# Autodesk Inventor assembly: gear_assembly
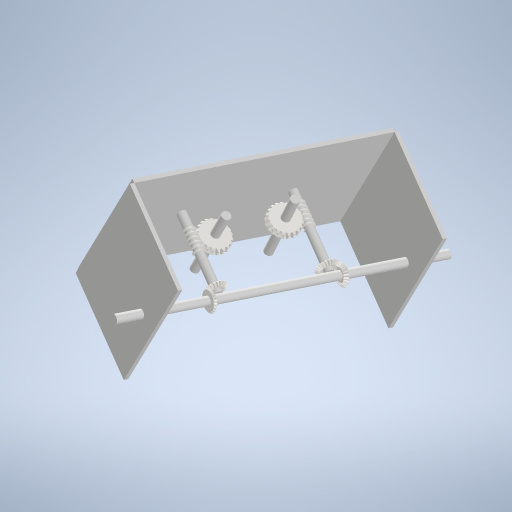
[picture p0: Inventor's stored thumbnail of the model, 512x512]
Saved by Autodesk Inventor 2023 (Build 270158000, 158)
## iProperties
Created: 2023-02-08
Part Number: gear_assembly
Document SubType Name: Assembly
Designer: Nikhil
Author: Nikhil
## Documents named in this file (8)
- C:\Users\Nikhil\Downloads\gear_assembly.iam
- C:\Users\Nikhil\Documents\ta202_autodesk\bridge\base_plate.ipt
- C:\Users\Nikhil\Documents\ta202_autodesk\bridge\shaft_120mm.ipt
- C:\Users\Nikhil\Documents\ta202_autodesk\bridge\assembly\Design Accelerator\Bevel Gears3.iam
- C:\Users\Nikhil\Documents\ta202_autodesk\bridge\assembly\Design Accelerator\Worm Gears1.iam
- C:\Users\Nikhil\Documents\ta202_autodesk\bridge\assembly\Design Accelerator\Worm Gears6.iam
- C:\Users\Nikhil\Documents\ta202_autodesk\bridge\rod_120mm.ipt
- C:\Users\Nikhil\Documents\ta202_autodesk\bridge\rod_450mm.ipt
## Components (11 placed, 6 different names)
1. base_plate:1 — Mate:1, Mate:2, Mate:3, Mate:4, Mate:7, Mate:11, Mate:18
2. shaft_120mm:1 — Mate:2, Mate:3, Mate:6, Mate:12
3. shaft_120mm:2 — Mate:1, Mate:4, Mate:10, Mate:13
4. Bevel Gears:3 [sub-assembly] — Mate:6, Mate:7, Mate:17
5. Worm Gears:1 [sub-assembly]
6. Bevel Gears:4 [sub-assembly] — Mate:10, Mate:11, Mate:16
7. Worm Gears:9 [sub-assembly] — Mate:12, Mate:14
8. Worm Gears:12 [sub-assembly] — Mate:13, Mate:15
9. rod_120mm:1 — Mate:14
10. rod_120mm:2 — Mate:15
11. rod_450mm:1 — Mate:16, Mate:17, Mate:18
## Relationships (15: Mate 15)
- Mate:1: base_plate:1 ↔ shaft_120mm:2
- Mate:2: base_plate:1 ↔ shaft_120mm:1
- Mate:3: base_plate:1 ↔ shaft_120mm:1
- Mate:4: base_plate:1 ↔ shaft_120mm:2
- Mate:6: shaft_120mm:1 ↔ Bevel Gears:3
- Mate:7: base_plate:1 ↔ Bevel Gears:3
- Mate:10: shaft_120mm:2 ↔ Bevel Gears:4
- Mate:11: base_plate:1 ↔ Bevel Gears:4
- Mate:12: shaft_120mm:1 ↔ Worm Gears:9
- Mate:13: shaft_120mm:2 ↔ Worm Gears:12
- Mate:14: Worm Gears:9 ↔ rod_120mm:1
- Mate:15: Worm Gears:12 ↔ rod_120mm:2
- Mate:16: Bevel Gears:4 ↔ rod_450mm:1
- Mate:17: Bevel Gears:3 ↔ rod_450mm:1
- Mate:18: base_plate:1 ↔ rod_450mm:1
